# Autodesk Inventor assembly: Ensamblaje1
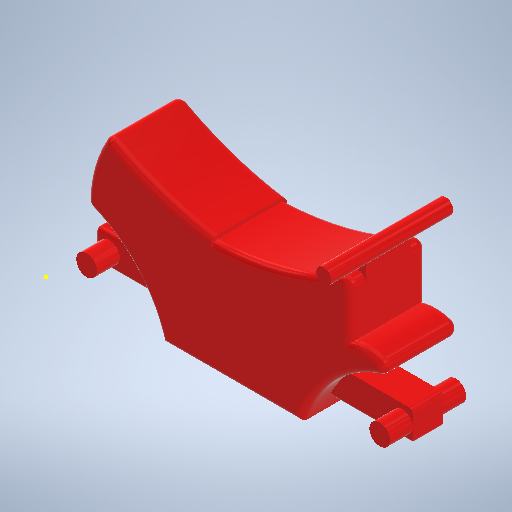
[picture p0: Inventor's stored thumbnail of the model, 512x512]
Saved by Autodesk Inventor 2025.2 (Build 292293000, 293)
## iProperties
Created: 2025-01-19
Part Number: Ensamblaje1
Document SubType Name: Assembly
Designer: usuario
Author: usuario
## Documents named in this file (3)
- C:\Users\usuario\Desktop\ModeladosAPM\MOTO\Ensamblaje1.iam
- C:\Users\usuario\Desktop\ModeladosAPM\MOTO\PiezaParteAtrasMoto.ipt
- C:\Users\usuario\Desktop\ModeladosAPM\MOTO\PiezaParteDelanteraMoto.ipt
## Components (2 placed, 2 different names)
1. PiezaParteAtrasMoto:1 — Coincidencia:1, Nivelación:1, Nivelación:2
2. PiezaParteDelanteraMoto:1 — Coincidencia:1, Nivelación:1, Nivelación:2
## Relationships (3: Flush 2, Mate 1)
- Coincidencia:1 [Mate]: PiezaParteAtrasMoto:1 ↔ PiezaParteDelanteraMoto:1
- Nivelación:1 [Flush]: PiezaParteAtrasMoto:1 ↔ PiezaParteDelanteraMoto:1
- Nivelación:2 [Flush]: PiezaParteAtrasMoto:1 ↔ PiezaParteDelanteraMoto:1
